# Autodesk Inventor assembly: X_CarriageR_V2_0
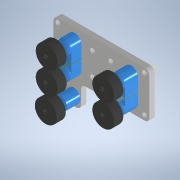
[picture p0: Inventor's stored thumbnail of the model, 180x180]
Saved by Autodesk Inventor 2021 (Build 250183000, 183)
## iProperties
Created: 2021-06-13
Part Number: X_CarriageR_V2_0
Document SubType Name: Assembly
Designer: Jorian Brusind
Author: Jorian Brusind
## Documents named in this file (7)
- C:\Users\Jorian Brusind\Documents\GitHub\PersonalProjects\HyperRail\Inventor Files\X_CarriageR_V2_0.iam
- C:\Users\Jorian Brusind\Documents\GitHub\PersonalProjects\HyperRail\Inventor Files\X_Carriage_Plate.ipt
- C:\Users\Jorian Brusind\Documents\GitHub\PersonalProjects\HyperRail\Inventor Files\11mm_BearingWheel.ipt
- C:\Users\Jorian Brusind\Documents\GitHub\PersonalProjects\HyperRail\Inventor Files\4mm_Roller_Spacer_simple.ipt
- C:\Users\Jorian Brusind\Documents\GitHub\PersonalProjects\HyperRail\Inventor Files\4mm_Roller_Spacer_simple3mm.ipt
- C:\Users\Jorian Brusind\Documents\GitHub\PersonalProjects\HyperRail\Inventor Files\Rollder_Spacer_Single.ipt
- C:\Users\Jorian Brusind\Documents\GitHub\PersonalProjects\HyperRail\Inventor Files\3mm_Spacer.ipt
## Components (10 placed, 6 different names)
1. X_Carriage_Plate:1 — Mate:1, Mate:2, Mate:3, Mate:5, Mate:8, Mate:9, Mate:13, Mate:24, Mate:25, Mate:26, Mate:35
2. 11mm_BearingWheel:1 — Mate:1, Mate:6, Flush:2
3. 11mm_BearingWheel:2 — Mate:5, Mate:6, Flush:1, Mate:11, Mate:36, Mate:39
4. 11mm_BearingWheel:3 — Mate:3, Mate:4, Flush:1, Flush:3, Mate:12, Flush:4
5. 11mm_BearingWheel:4 — Mate:2, Mate:4, Flush:2, Flush:3
6. 11mm_BearingWheel:5 — Mate:8, Mate:9, Flush:4, Mate:34, Mate:40
7. 4mm_Roller_Spacer_simple:1 — Mate:11, Mate:12, Mate:13
8. 4mm_Roller_Spacer_simple3mm:1 — Mate:24, Mate:25, Mate:26
9. Rollder_Spacer_Single:1 — Mate:34, Mate:35, Mate:40
10. 3mm_Spacer:1 — Mate:36, Mate:39
## Relationships (23: Mate 19, Flush 4)
- Mate:1: X_Carriage_Plate:1 ↔ 11mm_BearingWheel:1
- Mate:2: X_Carriage_Plate:1 ↔ 11mm_BearingWheel:4
- Mate:3 (2.75 mm): X_Carriage_Plate:1 ↔ 11mm_BearingWheel:3
- Mate:4 (62 mm): 11mm_BearingWheel:3 ↔ 11mm_BearingWheel:4
- Mate:5 (2.75 mm): X_Carriage_Plate:1 ↔ 11mm_BearingWheel:2
- Mate:6 (62 mm): 11mm_BearingWheel:1 ↔ 11mm_BearingWheel:2
- Flush:1: 11mm_BearingWheel:2 ↔ 11mm_BearingWheel:3
- Flush:2: 11mm_BearingWheel:1 ↔ 11mm_BearingWheel:4
- Flush:3: 11mm_BearingWheel:3 ↔ 11mm_BearingWheel:4
- Mate:8 (2.75 mm): X_Carriage_Plate:1 ↔ 11mm_BearingWheel:5
- Mate:9 (-10 mm): X_Carriage_Plate:1 ↔ 11mm_BearingWheel:5
- Mate:11: 11mm_BearingWheel:2 ↔ 4mm_Roller_Spacer_simple:1
- Mate:12: 11mm_BearingWheel:3 ↔ 4mm_Roller_Spacer_simple:1
- Mate:13: X_Carriage_Plate:1 ↔ 4mm_Roller_Spacer_simple:1
- Flush:4: 11mm_BearingWheel:3 ↔ 11mm_BearingWheel:5
- Mate:24: X_Carriage_Plate:1 ↔ 4mm_Roller_Spacer_simple3mm:1
- Mate:25: X_Carriage_Plate:1 ↔ 4mm_Roller_Spacer_simple3mm:1
- Mate:26: X_Carriage_Plate:1 ↔ 4mm_Roller_Spacer_simple3mm:1
- Mate:34: 11mm_BearingWheel:5 ↔ Rollder_Spacer_Single:1
- Mate:35: X_Carriage_Plate:1 ↔ Rollder_Spacer_Single:1
- Mate:36: 11mm_BearingWheel:2 ↔ 3mm_Spacer:1
- Mate:39: 11mm_BearingWheel:2 ↔ 3mm_Spacer:1
- Mate:40: 11mm_BearingWheel:5 ↔ Rollder_Spacer_Single:1
